# Autodesk Inventor assembly: przegub_1
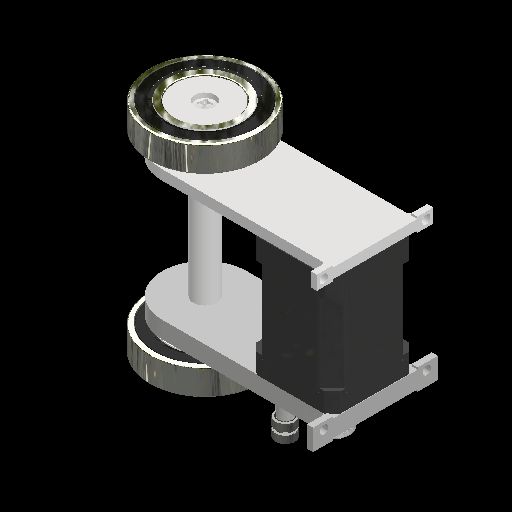
[picture p0: Inventor's stored thumbnail of the model, 512x512]
Saved by Autodesk Inventor 2024.4 (Build 284460000, 460)
## iProperties
Created: 2025-10-10
Part Number: przegub_1
Document SubType Name: Assembly
Designer: User
Mass: 189.382 g
Surface Area: 1021.35 cm^2
Volume: 189.382 cm^3
Density: 1 g/cm^3
Author: User
## Documents named in this file (18)
- C:\Users\Duszy\Desktop\Projekty\Dummy\Dummy_v2\Model\Model\przegub_2\przegub_1.iam
- C:\Users\Duszy\Desktop\Projekty\Dummy\Dummy_v2\Model\Model\przegub_2\24_zb_baza_v2 v1.ipt
- C:\Users\Duszy\Desktop\Projekty\Dummy\Dummy_v2\Model\Model\przegub_2\6661K89_Ball Bearing.ipt
- C:\Users\Duszy\Desktop\Projekty\Dummy\Dummy_v2\Model\Model\przegub_2\baza_rama_cz2.ipt
- C:\Users\Duszy\Desktop\Projekty\Dummy\Dummy_v2\Model\Model\przegub_2\connektor.ipt
- C:\Users\Duszy\Desktop\Projekty\Dummy\Dummy_v2\Model\Model\przegub_2\motor_1_rama.ipt
- C:\Users\Duszy\Desktop\Projekty\Dummy\Dummy_v2\Model\Model\przegub_2\NEMA 17 Stepper Motor 60mm-NEMA 17 Stepper Motor 60mm.ipt
- C:\Users\Duszy\Desktop\Projekty\Dummy\Dummy_v2\Model\Model\przegub_2\90258A189_Phillips Oval Head Screws.ipt
- C:\Users\Duszy\Desktop\Projekty\Dummy\Dummy_v2\Model\Model\przegub_2\94459A774_Heat-Set Inserts for Plastic.ipt
- C:\Users\Duszy\Desktop\Projekty\Dummy\Dummy_v2\Model\Model\przegub_2\90258A258_Phillips Oval Head Screws.ipt
- C:\Users\Duszy\Desktop\Projekty\Dummy\Dummy_v2\Model\Model\modele_gotowe\Modele_elementów\94459A150_Heat-Set Inserts for Plastic.ipt
- C:\Users\Duszy\Desktop\Projekty\Dummy\Dummy_v2\Model\Model\modele_gotowe\Modele_elementów\90258A218_Phillips Oval Head Screws.ipt
- C:\Users\Duszy\Desktop\Projekty\Dummy\Dummy_v2\Model\Model\przegub_2\7804K106_Stainless Steel Ball Bearing.ipt
- C:\Users\Duszy\Desktop\Projekty\Dummy\Dummy_v2\Model\Model\przegub_2\przegub_1\AIP\FEA\f7pdpprs0.fins
- C:\Users\Duszy\Desktop\Projekty\Dummy\Dummy_v2\Model\Model\przegub_2\przegub_1\AIP\FEA\f7pdpprsw.fsat
- C:\Users\Duszy\Desktop\Projekty\Dummy\Dummy_v2\Model\Model\przegub_2\przegub_1\AIP\FEA\f7pdpprsw.ftes
- C:\Users\Duszy\Desktop\Projekty\Dummy\Dummy_v2\Model\Model\przegub_2\przegub_1\AIP\FEA\f7pdpprsw.fwiz
- C:\Users\Duszy\Desktop\Projekty\Dummy\Dummy_v2\Model\Model\przegub_2\przegub_1\AIP\FEA\f7pdpps4g.fmsh
## Components (21 placed, 12 different names)
1. 24_zb_baza_v2 v1:1 — Obrotowe:2, Obrotowe:11
2. 6661K89_Ball Bearing:1 — Obrotowe:1
3. baza_rama_cz2:1 — Obrotowe:3, Obrotowe:4
4. connektor:1 — Sztywne:2, Obrotowe:3, Sztywne:3, Obrotowe:7
5. motor_1_rama:1 — Obrotowe:1, Sztywne:2, Obrotowe:12, Obrotowe:14, Obrotowe:15
6. NEMA 17 Stepper Motor 60mm-NEMA 17 Stepper Motor 60mm:1 — Obrotowe:2, Obrotowe:12, Obrotowe:13
7. 6661K89_Ball Bearing:2 — Obrotowe:4
8. 94459A774_Heat-Set Inserts for Plastic:1 — Sztywne:3, Obrotowe:9
9. 94459A774_Heat-Set Inserts for Plastic:2 — Obrotowe:7, Obrotowe:8
10. 90258A258_Phillips Oval Head Screws:1 — Obrotowe:8
11. 90258A258_Phillips Oval Head Screws:2 — Obrotowe:9
12. 94459A150_Heat-Set Inserts for Plastic:1 — Obrotowe:10, Obrotowe:11
13. 90258A218_Phillips Oval Head Screws:1 — Obrotowe:10
14. 90258A189_Phillips Oval Head Screws:3 — Obrotowe:13
15. 90258A189_Phillips Oval Head Screws:4
16. 90258A189_Phillips Oval Head Screws:5
17. 90258A189_Phillips Oval Head Screws:6
18. 7804K106_Stainless Steel Ball Bearing:3 — Obrotowe:14
19. 7804K106_Stainless Steel Ball Bearing:2 — Obrotowe:15
20. 7804K106_Stainless Steel Ball Bearing:4
21. 7804K106_Stainless Steel Ball Bearing:5
## Component patterns: (4 elements, first: 90258A189_Phillips Oval Head Screws:3), (2 elements, first: 7804K106_Stainless Steel Ball Bearing:3 + 7804K106_Stainless Steel Ball Bearing:2)
## Relationships (15: RevoluteJoint 13, WeldJoint 2)
- Obrotowe:1 [RevoluteJoint] (-11 mm): 6661K89_Ball Bearing:1 ↔ motor_1_rama:1
- Obrotowe:2 [RevoluteJoint]: 24_zb_baza_v2 v1:1 ↔ NEMA 17 Stepper Motor 60mm-NEMA 17 Stepper Motor 60mm:1
- Sztywne:2 [WeldJoint]: connektor:1 ↔ motor_1_rama:1
- Obrotowe:3 [RevoluteJoint]: baza_rama_cz2:1 ↔ connektor:1
- Obrotowe:4 [RevoluteJoint] (-12 mm): baza_rama_cz2:1 ↔ 6661K89_Ball Bearing:2
- Sztywne:3 [WeldJoint] (-5.7 mm): connektor:1 ↔ 94459A774_Heat-Set Inserts for Plastic:1
- Obrotowe:7 [RevoluteJoint] (5.7 mm): connektor:1 ↔ 94459A774_Heat-Set Inserts for Plastic:2
- Obrotowe:8 [RevoluteJoint] (-8 mm): 94459A774_Heat-Set Inserts for Plastic:2 ↔ 90258A258_Phillips Oval Head Screws:1
- Obrotowe:9 [RevoluteJoint] (-8 mm): 94459A774_Heat-Set Inserts for Plastic:1 ↔ 90258A258_Phillips Oval Head Screws:2
- Obrotowe:10 [RevoluteJoint] (9 mm): 94459A150_Heat-Set Inserts for Plastic:1 ↔ 90258A218_Phillips Oval Head Screws:1
- Obrotowe:11 [RevoluteJoint] (-0.9 mm): 24_zb_baza_v2 v1:1 ↔ 94459A150_Heat-Set Inserts for Plastic:1
- Obrotowe:12 [RevoluteJoint] (-8.4 mm): motor_1_rama:1 ↔ NEMA 17 Stepper Motor 60mm-NEMA 17 Stepper Motor 60mm:1
- Obrotowe:13 [RevoluteJoint] (-11 mm): NEMA 17 Stepper Motor 60mm-NEMA 17 Stepper Motor 60mm:1 ↔ 90258A189_Phillips Oval Head Screws:3
- Obrotowe:14 [RevoluteJoint] (-5 mm): motor_1_rama:1 ↔ 7804K106_Stainless Steel Ball Bearing:3
- Obrotowe:15 [RevoluteJoint]: motor_1_rama:1 ↔ 7804K106_Stainless Steel Ball Bearing:2
## Named parameters: sa_0 = 20000, sa_1 = 20000
note: some values were not read from the file. Shown as the stored number, unit unknown: "sa_0", "sa_1".
